# Autodesk Inventor assembly: Vex Wheel Assembly
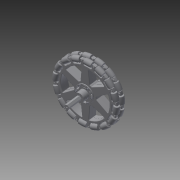
[picture p0: Inventor's stored thumbnail of the model, 180x180]
Saved by Autodesk Inventor 2013 (Build 170138000, 138)
## iProperties
Created: 2013-01-10
Part Number: Vex Wheel Assembly
Document SubType Name: Assembly
Designer: Naphat
Author: Naphat
## Documents named in this file (7)
- C:\Users\carneeki\Desktop\Kiwi Robot\Vex Wheel\Vex Wheel Assembly.iam
- C:\Users\carneeki\Desktop\Kiwi Robot\Imported Components\217-2613.20121203\217-2613.20121203.iam
- C:\Users\carneeki\Desktop\Kiwi Robot\217-2592.20121203.ipt
- C:\Users\carneeki\Desktop\Kiwi Robot\Hex Shaft.ipt
- C:\Users\carneeki\Desktop\Kiwi Robot\Vex Wheel\ShaftCollar.ipt
- C:\Users\carneeki\Documents\Inventor\Content Center Files\R2013\en-US\ANSI B18.3(05)\ANSI B18.3 - 8-32 UNC - 1.5(31).ipt
- C:\Users\carneeki\Documents\Inventor\Content Center Files\R2013\en-US\IFI 100 107(2)\IFI 100_107 - No. 8 - 32 Top Insert Type.ipt
## Components (17 placed, 6 different names)
1. 217-2613.20121203:1 [sub-assembly] — Insert:7, Insert:8, Insert:9, Insert:10, Insert:11, Insert:12
2. 217-2592.20121203:1 — Mate:1, Mate:2, Mate:4, Insert:1, Insert:2, Insert:3, Insert:4, Insert:5, Insert:6
3. Hex Shaft:1 — Mate:1, Mate:3, Mate:7, Mate:8, Mate:9
4. ShaftCollar:1 — Mate:3, Mate:4
5. ShaftCollar:2 — Mate:2, Mate:7, Mate:8, Mate:9
6. Hexagon Socket Head Cap Screw - Inch No. 8 - 32 UNC - 1 1/2:1 — Insert:1
7. Hexagon Socket Head Cap Screw - Inch No. 8 - 32 UNC - 1 1/2:2 — Insert:2
8. Hexagon Socket Head Cap Screw - Inch No. 8 - 32 UNC - 1 1/2:3 — Insert:3
9. Hexagon Socket Head Cap Screw - Inch No. 8 - 32 UNC - 1 1/2:4 — Insert:4
10. Hexagon Socket Head Cap Screw - Inch No. 8 - 32 UNC - 1 1/2:5 — Insert:5
11. Hexagon Socket Head Cap Screw - Inch No. 8 - 32 UNC - 1 1/2:6 — Insert:6
12. Prevailing Torque Type Hex Nut - Inch (IFI) No. 8 - 32 Top Insert Type:1 — Insert:7
13. Prevailing Torque Type Hex Nut - Inch (IFI) No. 8 - 32 Top Insert Type:2 — Insert:8
14. Prevailing Torque Type Hex Nut - Inch (IFI) No. 8 - 32 Top Insert Type:3 — Insert:9
15. Prevailing Torque Type Hex Nut - Inch (IFI) No. 8 - 32 Top Insert Type:4 — Insert:10
16. Prevailing Torque Type Hex Nut - Inch (IFI) No. 8 - 32 Top Insert Type:5 — Insert:11
17. Prevailing Torque Type Hex Nut - Inch (IFI) No. 8 - 32 Top Insert Type:6 — Insert:12
## Relationships (19: Insert 12, Mate 7)
- Mate:1: 217-2592.20121203:1 ↔ Hex Shaft:1
- Mate:2: 217-2592.20121203:1 ↔ ShaftCollar:2
- Mate:3: Hex Shaft:1 ↔ ShaftCollar:1
- Mate:4: 217-2592.20121203:1 ↔ ShaftCollar:1
- Mate:7: Hex Shaft:1 ↔ ShaftCollar:2
- Mate:8: Hex Shaft:1 ↔ ShaftCollar:2
- Mate:9: Hex Shaft:1 ↔ ShaftCollar:2
- Insert:1: 217-2592.20121203:1 ↔ Hexagon Socket Head Cap Screw - Inch No. 8 - 32 UNC - 1 1/2:1
- Insert:2: 217-2592.20121203:1 ↔ Hexagon Socket Head Cap Screw - Inch No. 8 - 32 UNC - 1 1/2:2
- Insert:3: 217-2592.20121203:1 ↔ Hexagon Socket Head Cap Screw - Inch No. 8 - 32 UNC - 1 1/2:3
- Insert:4: 217-2592.20121203:1 ↔ Hexagon Socket Head Cap Screw - Inch No. 8 - 32 UNC - 1 1/2:4
- Insert:5: 217-2592.20121203:1 ↔ Hexagon Socket Head Cap Screw - Inch No. 8 - 32 UNC - 1 1/2:5
- Insert:6: 217-2592.20121203:1 ↔ Hexagon Socket Head Cap Screw - Inch No. 8 - 32 UNC - 1 1/2:6
- Insert:7: 217-2613.20121203:1 ↔ Prevailing Torque Type Hex Nut - Inch (IFI) No. 8 - 32 Top Insert Type:1
- Insert:8: 217-2613.20121203:1 ↔ Prevailing Torque Type Hex Nut - Inch (IFI) No. 8 - 32 Top Insert Type:2
- Insert:9: 217-2613.20121203:1 ↔ Prevailing Torque Type Hex Nut - Inch (IFI) No. 8 - 32 Top Insert Type:3
- Insert:10: 217-2613.20121203:1 ↔ Prevailing Torque Type Hex Nut - Inch (IFI) No. 8 - 32 Top Insert Type:4
- Insert:11: 217-2613.20121203:1 ↔ Prevailing Torque Type Hex Nut - Inch (IFI) No. 8 - 32 Top Insert Type:5
- Insert:12: 217-2613.20121203:1 ↔ Prevailing Torque Type Hex Nut - Inch (IFI) No. 8 - 32 Top Insert Type:6
